# Autodesk Inventor assembly: Shoulder_support_assembly
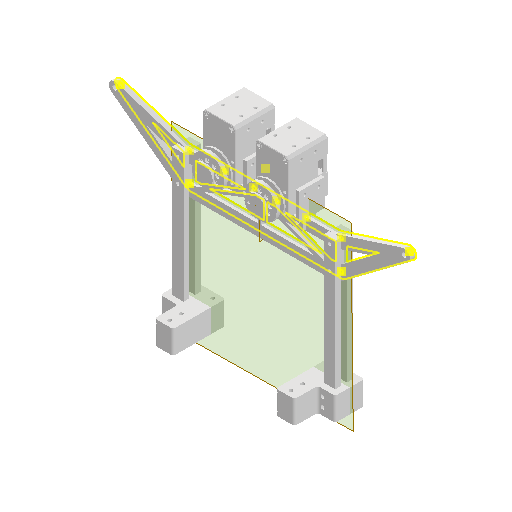
[picture p0: Inventor's stored thumbnail of the model, 512x512]
Saved by Autodesk Inventor 2022 (Build 260153000, 153)
## iProperties
Created: 2022-08-23
Part Number: Shoulder_support_assembly
Document SubType Name: Assembly
Designer: dell
Mass: 102.221 g
Surface Area: 678.671 cm^2
Volume: 102.221 cm^3
Density: 1 g/cm^3
Author: dell
## Documents named in this file (5)
- D:\xxxx\Uni\Part IV\MECHENG_700\Part_IV_project_CAD\Bird_skeleton_prototypes\Wing_drone_V1\Bird_wing_V2\Wing_shoulder\Shoulder_support_assembly.iam
- D:\xxxx\Uni\Part IV\MECHENG_700\Part_IV_project_CAD\Bird_skeleton_prototypes\Wing_drone_V1\Bird_wing_V2\Wing_shoulder\Vertical_bar.ipt
- D:\xxxx\Uni\Part IV\MECHENG_700\Part_IV_project_CAD\Bird_skeleton_prototypes\Wing_drone_V1\Bird_wing_V2\Wing_shoulder\Bar_connection_assembly.iam
- D:\xxxx\Uni\Part IV\MECHENG_700\Part_IV_project_CAD\Bird_skeleton_prototypes\Wing_drone_V1\Bird_wing_V2\Wing_shoulder\Horizontal_bar_V2.ipt
- D:\xxxx\Uni\Part IV\MECHENG_700\Part_IV_project_CAD\Bird_skeleton_prototypes\Wing_drone_V1\Bird_wing_V2\Motor_pulley_assembly.iam
## Components (9 placed, 4 different names)
1. Vertical_bar:1 — Flush:1, Flush:4, Mate:5, Symmetry:1, Mate:12
2. Vertical_bar:2 — Flush:1, Flush:4, Mate:9, Mate:10, Flush:8, Mate:12, Mate:13, Mate:17
3. Vertical_bar:3 — Flush:2, Flush:3, Symmetry:1, Mate:7, Mate:8, Flush:7, Mate:15, Mate:18
4. Vertical_bar:4 — Flush:2, Flush:3, Mate:5, Mate:16
5. Bar_connection_assembly:1 [sub-assembly] — Mate:9, Mate:10, Flush:8
6. Bar_connection_assembly:2 [sub-assembly] — Mate:7, Mate:8, Flush:7
7. Horizontal_bar_V2:1 — Mate:13, Mate:15, Mate:16, Mate:17, Mate:18, Mate:19, Mate:20, Mate:21, Mate:23, Mate:24, Mate:25
8. Motor_pulley_assembly:3 [sub-assembly] — Mate:19, Mate:20, Mate:21, Mate:22
9. Motor_pulley_assembly:4 [sub-assembly] — Mate:23, Mate:24, Mate:25
## Relationships (25: Mate 18, Flush 6, Symmetry 1)
- Flush:1: Vertical_bar:1 ↔ Vertical_bar:2
- Flush:2: Vertical_bar:3 ↔ Vertical_bar:4
- Flush:3: Vertical_bar:3 ↔ Vertical_bar:4
- Flush:4: Vertical_bar:1 ↔ Vertical_bar:2
- Mate:5 (120 mm): Vertical_bar:1 ↔ Vertical_bar:4
- Symmetry:1: Vertical_bar:1 ↔ Vertical_bar:3
- Mate:7: Vertical_bar:3 ↔ Bar_connection_assembly:2
- Mate:8: Vertical_bar:3 ↔ Bar_connection_assembly:2
- Flush:7: Vertical_bar:3 ↔ Bar_connection_assembly:2
- Mate:9: Vertical_bar:2 ↔ Bar_connection_assembly:1
- Mate:10: Vertical_bar:2 ↔ Bar_connection_assembly:1
- Flush:8: Vertical_bar:2 ↔ Bar_connection_assembly:1
- Mate:12 (5 mm): Vertical_bar:1 ↔ Vertical_bar:2
- Mate:13: Vertical_bar:2 ↔ Horizontal_bar_V2:1
- Mate:15: Vertical_bar:3 ↔ Horizontal_bar_V2:1
- Mate:16: Vertical_bar:4 ↔ Horizontal_bar_V2:1
- Mate:17: Vertical_bar:2 ↔ Horizontal_bar_V2:1
- Mate:18: Vertical_bar:3 ↔ Horizontal_bar_V2:1
- Mate:19: Horizontal_bar_V2:1 ↔ Motor_pulley_assembly:3
- Mate:20: Horizontal_bar_V2:1 ↔ Motor_pulley_assembly:3
- Mate:21: Horizontal_bar_V2:1 ↔ Motor_pulley_assembly:3
- Mate:22: Motor_pulley_assembly:3
- Mate:23: Horizontal_bar_V2:1 ↔ Motor_pulley_assembly:4
- Mate:24: Horizontal_bar_V2:1 ↔ Motor_pulley_assembly:4
- Mate:25: Horizontal_bar_V2:1 ↔ Motor_pulley_assembly:4
